# Autodesk Inventor assembly: Final
(part 3 of 3)
- Mate:825: Cap_Platine:3 ↔ din_en_iso_4762_m3x6:5
- Mate:826: Cap_Platine:3 ↔ din_en_iso_4762_m3x6:8
- Mate:827: Cap_Platine:2 ↔ din_en_iso_4762_m3x6:10
- Mate:828: Cap_Platine:2 ↔ din_en_iso_4762_m3x6:15
- Mate:829: Cap_Platine:1 ↔ din_en_iso_4762_m3x6:14
- Mate:830: Cap_Platine:1 ↔ din_en_iso_4762_m3x6:7
- Mate:831: Cap_Platine:6 ↔ din_en_iso_4762_m3x6:3
- Mate:832: Cap_Platine:6 ↔ din_en_iso_4762_m3x6:2
- Mate:833: Cap_Platine:1 ↔ din_en_iso_4762_m3x6:18
- Mate:834: Cap_Platine:4 ↔ din_en_iso_4762_m3x6:16
- Mate:835: Cap_Platine:2 ↔ din_en_iso_4762_m3x6:17
- Mate:836: Cap_Platine:6 ↔ din_en_iso_4762_m3x6:11
- Mate:837: Cap_Platine:3 ↔ din_en_iso_4762_m3x6:13
- Mate:838: Cap_Platine:4 ↔ din_en_iso_4762_m3x6:12
- Mate:839: Cap_Platine:4 ↔ din_en_iso_4762_m3x6:4
- Mate:840: Cap_Platine:3 ↔ din_en_iso_4762_m3x6:8
- Mate:841: Cap_Platine:3 ↔ din_en_iso_4762_m3x6:5
- Mate:842: Secondary:1 ↔ PrimaryCoil:1
- Mate:843: primary_holder:6 ↔ PrimaryCoil:1
- Mate:844: SeitenUnten:2 ↔ Lüfter:4
- Mate:845: SeitenUnten:2 ↔ Lüfter:3
- Mate:846: SeitenUnten:1 ↔ Lüfter:2
- Mate:847: SeitenUnten:1 ↔ Lüfter:1
- Mate:848: SeitenUnten:1 ↔ Lüfter:2
- Mate:849: SeitenUnten:1 ↔ Lüfter:1
- Mate:850: SeitenUnten:2 ↔ Lüfter:3
- Mate:851: SeitenUnten:2 ↔ Lüfter:4
- Mate:852: SeitenUnten:2 ↔ Lüfter:3
- Mate:853: SeitenUnten:2 ↔ Lüfter:4
- Mate:854: SeitenUnten:1 ↔ Lüfter:2
- Mate:855: SeitenUnten:1 ↔ Lüfter:1
- Mate:887: Heatsink:1 ↔ Abstandshalter_5mm:5
- Mate:888: Heatsink:1 ↔ Abstandshalter_5mm:2
- Mate:889: Heatsink:1 ↔ Abstandshalter_5mm:3
- Mate:890: Heatsink:1 ↔ Abstandshalter_5mm:1
- Mate:891: Heatsink:1 ↔ Abstandshalter_5mm:6
- Mate:892: Heatsink:1 ↔ Abstandshalter_5mm:4
- Mate:893: Heatsink:1 ↔ Abstandshalter_5mm:2
- Mate:894: Heatsink:1 ↔ Abstandshalter_5mm:3
- Mate:895: Heatsink:1 ↔ Abstandshalter_5mm:1
- Mate:896: Heatsink:1 ↔ Abstandshalter_5mm:5
- Mate:897: Heatsink:1 ↔ Abstandshalter_5mm:6
- Mate:898: Heatsink:1 ↔ Abstandshalter_5mm:4
- Mate:899: Abstandshalter_5mm:2 ↔ GDT:2
- Mate:900: Abstandshalter_5mm:1 ↔ GDT:1
- Mate:901: Abstandshalter_5mm:4 ↔ GDT:1
- Mate:902: Abstandshalter_5mm:3 ↔ GDT:1
- Mate:903: Abstandshalter_5mm:2 ↔ GDT:2
- Mate:904: Abstandshalter_5mm:6 ↔ GDT:2
- Mate:905: GDT:2 ↔ din_en_iso_4762_m3x6:21
- Mate:906: GDT:2 ↔ din_en_iso_4762_m3x6:20
- Mate:907: GDT:2 ↔ din_en_iso_4762_m3x6:23
- Mate:908: GDT:1 ↔ din_en_iso_4762_m3x6:24
- Mate:909: GDT:1 ↔ din_en_iso_4762_m3x6:19
- Mate:910: GDT:1 ↔ din_en_iso_4762_m3x6:22
- Mate:911: GDT:1 ↔ din_en_iso_4762_m3x6:19
- Mate:912: GDT:1 ↔ din_en_iso_4762_m3x6:22
- Mate:913: GDT:1 ↔ din_en_iso_4762_m3x6:24
- Mate:914: GDT:2 ↔ din_en_iso_4762_m3x6:23
- Mate:915: GDT:2 ↔ din_en_iso_4762_m3x6:21
- Mate:916: GDT:2 ↔ din_en_iso_4762_m3x6:20
- Mate:917: bottom:1 ↔ LogicHolder:1
- Mate:923: SeitenUntenHinten:1 ↔ din_en_iso_4762_m3x10:16
- Mate:924: SeitenUntenHinten:1 ↔ din_en_iso_4762_m3x10:15
- Mate:925: SeitenUntenHinten:1 ↔ din_en_iso_4762_m3x10:16
- Mate:926: SeitenUntenHinten:1 ↔ din_en_iso_4762_m3x10:15
- Mate:927: Netzstecker:1 ↔ din_en_iso_7991_m3x10:4
- Mate:928: Netzstecker:1 ↔ din_en_iso_7991_m3x10:2
- Mate:929: Netzstecker:2 ↔ din_en_iso_7991_m3x10:3
- Mate:930: Netzstecker:2 ↔ din_en_iso_7991_m3x10:1
- Flush:480: Netzstecker:1 ↔ din_en_iso_7991_m3x10:2
- Flush:481: Netzstecker:1 ↔ din_en_iso_7991_m3x10:4
- Flush:482: Netzstecker:2 ↔ din_en_iso_7991_m3x10:1
- Flush:483: Netzstecker:2 ↔ din_en_iso_7991_m3x10:3
- Mate:932: LogicHolder:1 ↔ din_en_iso_7991_m3x10:5
- Mate:933: LogicHolder:1 ↔ din_en_iso_7991_m3x10:6
- Mate:934: bottom:1 ↔ NtHolder:1
- Mate:936: NtHolder:1 ↔ Power_Supply_S_90_18:1
- Mate:937: NtHolder:1 ↔ Power_Supply_S_90_18:1
- Mate:938: NtHolder:1 ↔ din_en_iso_7991_m3x10:8
- Mate:939: NtHolder:1 ↔ din_en_iso_7991_m3x10:7
- Mate:940: NtHolder:1 ↔ din_en_iso_7991_m3x10:9
- Mate:941: NtHolder:1 ↔ din_en_iso_7991_m3x10:10
- Flush:484: LogicHolder:1 ↔ din_en_iso_7991_m3x10:5
- Flush:485: LogicHolder:1 ↔ din_en_iso_7991_m3x10:6
- Flush:486: NtHolder:1 ↔ din_en_iso_7991_m3x10:10
- Flush:487: NtHolder:1 ↔ din_en_iso_7991_m3x10:9
- Flush:488: NtHolder:1 ↔ din_en_iso_7991_m3x10:8
- Flush:489: NtHolder:1 ↔ din_en_iso_7991_m3x10:7
- Mate:942: din_en_iso_7991_m3x10:1 ↔ mutter_din934_m3-6:25
- Mate:943: SeitenUntenHinten:1 ↔ mutter_din934_m3-6:25
- Mate:944: din_en_iso_4762_m3x10:15 ↔ mutter_din934_m3-6:27
- Mate:945: din_en_iso_7991_m3x10:3 ↔ mutter_din934_m3-6:26
- Mate:946: SeitenUntenHinten:1 ↔ mutter_din934_m3-6:26
- Mate:947: Netzfilter:1 ↔ mutter_din934_m3-6:27
- Mate:948: din_en_iso_7991_m3x10:2 ↔ mutter_din934_m3-6:24
- Mate:949: SeitenUntenHinten:1 ↔ mutter_din934_m3-6:24
- Mate:950: din_en_iso_7991_m3x10:4 ↔ mutter_din934_m3-6:28
- Mate:951: din_en_iso_4762_m3x10:16 ↔ mutter_din934_m3-6:23
- Mate:952: Netzfilter:1 ↔ mutter_din934_m3-6:23
- Mate:953: SeitenUntenHinten:1 ↔ mutter_din934_m3-6:28
- Mate:954: Lüfter:2 ↔ din_en_iso_7991_m4x35:16
- Mate:955: Lüfter:1 ↔ din_en_iso_7991_m4x35:9
- Mate:956: Lüfter:1 ↔ din_en_iso_7991_m4x35:10
- Mate:957: Lüfter:2 ↔ din_en_iso_7991_m4x35:11
- Mate:958: Lüfter:2 ↔ din_en_iso_7991_m4x35:12
- Mate:959: Lüfter:2 ↔ din_en_iso_7991_m4x35:13
- Mate:960: Lüfter:1 ↔ din_en_iso_7991_m4x35:14
- Mate:961: Lüfter:1 ↔ din_en_iso_7991_m4x35:15
- Mate:962: Lüfter:4 ↔ din_en_iso_7991_m4x35:1
- Mate:963: Lüfter:4 ↔ din_en_iso_7991_m4x35:2
- Mate:964: Lüfter:4 ↔ din_en_iso_7991_m4x35:3
- Mate:965: Lüfter:4 ↔ din_en_iso_7991_m4x35:4
- Mate:966: Lüfter:3 ↔ din_en_iso_7991_m4x35:5
- Mate:967: Lüfter:3 ↔ din_en_iso_7991_m4x35:6
- Mate:968: Lüfter:3 ↔ din_en_iso_7991_m4x35:7
- Mate:969: Lüfter:3 ↔ din_en_iso_7991_m4x35:8
- Flush:490: SeitenUnten:1 ↔ din_en_iso_7991_m4x35:9
- Flush:491: SeitenUnten:1 ↔ din_en_iso_7991_m4x35:10
- Flush:971: SeitenUnten:1 ↔ din_en_iso_7991_m4x35:11
- Flush:492: SeitenUnten:1 ↔ din_en_iso_7991_m4x35:15
- Flush:493: SeitenUnten:1 ↔ din_en_iso_7991_m4x35:12
- Flush:494: SeitenUnten:1 ↔ din_en_iso_7991_m4x35:13
- Flush:495: SeitenUnten:1 ↔ din_en_iso_7991_m4x35:16
- Flush:496: SeitenUnten:1 ↔ din_en_iso_7991_m4x35:14
- Mate:971: din_en_iso_7991_m4x35:9 ↔ mutter_din934_m4-10:33
- Mate:972: din_en_iso_7991_m4x35:10 ↔ mutter_din934_m4-10:27
- Mate:973: din_en_iso_7991_m4x35:15 ↔ mutter_din934_m4-10:30
- Mate:974: din_en_iso_7991_m4x35:12 ↔ mutter_din934_m4-10:29
- Mate:975: din_en_iso_7991_m4x35:13 ↔ mutter_din934_m4-10:28
- Mate:976: din_en_iso_7991_m4x35:16 ↔ mutter_din934_m4-10:32
- Mate:977: din_en_iso_7991_m4x35:14 ↔ mutter_din934_m4-10:34
- Mate:986: din_en_iso_7991_m4x35:11 ↔ mutter_din934_m4-10:31
- Mate:988: Schalter:1 ↔ Rändelmutter:1
- Mate:989: SeitenUntenVorne:1 ↔ Rändelmutter:1
- Mate:990: Schalter:2 ↔ Rändelmutter:2
- Mate:991: SeitenUntenVorne:1 ↔ Rändelmutter:2
- Flush:972: SeitenUnten:2 ↔ din_en_iso_7991_m4x35:7
- Flush:973: SeitenUnten:2 ↔ din_en_iso_7991_m4x35:8
- Flush:974: SeitenUnten:2 ↔ din_en_iso_7991_m4x35:1
- Flush:975: SeitenUnten:2 ↔ din_en_iso_7991_m4x35:6
- Flush:976: SeitenUnten:2 ↔ din_en_iso_7991_m4x35:2
- Flush:993: SeitenUnten:2 ↔ din_en_iso_7991_m4x35:5
- Mate:992: din_en_iso_7991_m4x35:7 ↔ mutter_din934_m4-10:41
- Mate:994: din_en_iso_7991_m4x35:1 ↔ mutter_din934_m4-10:38
- Mate:996: din_en_iso_7991_m4x35:8 ↔ mutter_din934_m4-10:37
- Mate:997: din_en_iso_7991_m4x35:2 ↔ mutter_din934_m4-10:36
- Mate:1000: din_en_iso_7991_m4x35:6 ↔ mutter_din934_m4-10:42
- Mate:1001: din_en_iso_7991_m4x35:5 ↔ mutter_din934_m4-10:39
- Flush:994: SeitenUnten:2 ↔ din_en_iso_7991_m4x35:4
- Flush:995: SeitenUnten:2 ↔ din_en_iso_7991_m4x35:3
- Mate:1002: din_en_iso_7991_m4x35:3 ↔ mutter_din934_m4-10:40
- Mate:1004: din_en_iso_7991_m4x35:4 ↔ mutter_din934_m4-10:35
- Mate:1007: mid:1 ↔ CT_Holder:2
- Mate:1008: mid:1 ↔ CT_Holder:1
- Angle:7 (0 deg): mid:1 ↔ CT_Holder:1
- Angle:8 (0 deg): mid:1 ↔ CT_Holder:2
- [Mate]: mid:1 ↔ din_en_iso_4762_m3x10:18
- [Mate]: mid:1 ↔ din_en_iso_4762_m3x10:17
- Mate:1011: din_en_iso_4762_m3x10:18 ↔ mutter_din934_m3-6:30
- Mate:1012: mid:1 ↔ mutter_din934_m3-6:30
- Mate:1013: din_en_iso_4762_m3x10:17 ↔ mutter_din934_m3-6:29
- Mate:1014: mid:1 ↔ mutter_din934_m3-6:29
- Mate:1015: Platine_Gleichrichter:1 ↔ din125-1-a_5_3-140_hv:1
- Mate:1016: Cu_Cap:2 ↔ din_en_iso_4762_m5x10:3
- Mate:1017: Cu_Cap:1 ↔ din_en_iso_4762_m5x10:7
- Mate:1018: din125-1-a_5_3-140_hv:6 ↔ din_en_iso_4762_m5x10:2
- Mate:1019: din125-1-a_5_3-140_hv:11 ↔ din_en_iso_4762_m5x10:4
- Mate:1020: din125-1-a_5_3-140_hv:7 ↔ din_en_iso_4762_m5x10:2
- Mate:1021: din125-1-a_5_3-140_hv:5 ↔ din_en_iso_4762_m5x10:4
- Mate:1022: din125-1-a_5_3-140_hv:8 ↔ din_en_iso_4762_m5x10:5
- Mate:1023: din125-1-a_5_3-140_hv:9 ↔ din_en_iso_4762_m5x10:5
- Mate:1024: din125-1-a_5_3-140_hv:10 ↔ din_en_iso_4762_m5x10:8
- Mate:1025: din125-1-a_5_3-140_hv:12 ↔ din_en_iso_4762_m5x10:8
- Mate:1026: din125-1-a_5_3-140_hv:5 ↔ din125-1-a_5_3-140_hv:11
- Mate:1027: Cu_Cap:2 ↔ din125-1-a_5_3-140_hv:11
- Mate:1028: din125-1-a_5_3-140_hv:6 ↔ din125-1-a_5_3-140_hv:7
- Mate:1029: Cu_Cap:1 ↔ din125-1-a_5_3-140_hv:7
- Mate:1030: din125-1-a_5_3-140_hv:8 ↔ din125-1-a_5_3-140_hv:9
- Mate:1031: Cu_Cap:1 ↔ din125-1-a_5_3-140_hv:8
- Mate:1032: din125-1-a_5_3-140_hv:10 ↔ din125-1-a_5_3-140_hv:12
- Mate:1033: Cu_Cap:2 ↔ din125-1-a_5_3-140_hv:12
- Mate:1034: din125-1-a_5_3-140_hv:14 ↔ din_en_iso_4762_m5x10:4
- Mate:1035: din125-1-a_5_3-140_hv:16 ↔ din_en_iso_4762_m5x10:2
- Mate:1036: din125-1-a_5_3-140_hv:5 ↔ din125-1-a_5_3-140_hv:14
- Mate:1037: din125-1-a_5_3-140_hv:6 ↔ din125-1-a_5_3-140_hv:16
- Mate:1038: din125-1-a_5_3-140_hv:13 ↔ din_en_iso_4762_m5x10:5
- Mate:1039: din125-1-a_5_3-140_hv:15 ↔ din_en_iso_4762_m5x10:8
- Mate:1040: din125-1-a_5_3-140_hv:10 ↔ din125-1-a_5_3-140_hv:15
- Mate:1041: din125-1-a_5_3-140_hv:9 ↔ din125-1-a_5_3-140_hv:13
- Mate:1042: Cap:2 ↔ din125-1-a_5_3-140_hv:16
- Mate:1043: din_en_iso_4762_m5x10:7 ↔ mutter_din934_m5-6:11
- Mate:1044: din_en_iso_4762_m5x10:3 ↔ mutter_din934_m5-6:12
- Mate:1045: Cu_Cap:1 ↔ mutter_din934_m5-6:11
- Mate:1046: Cu_Cap:2 ↔ mutter_din934_m5-6:12
- Mate:1047: Lüftergitter:4 ↔ Lüfter:2
- Mate:1048: Lüftergitter:3 ↔ Lüfter:1
- Mate:1049: Lüftergitter:4 ↔ din_en_iso_7991_m4x35:16
- Mate:1050: Lüftergitter:4 ↔ din_en_iso_7991_m4x35:13
- Mate:1051: Lüftergitter:4 ↔ mutter_din934_m4-10:32
- Mate:1052: Lüftergitter:4 ↔ mutter_din934_m4-10:28
- Mate:1053: Lüftergitter:3 ↔ din_en_iso_7991_m4x35:10
- Mate:1054: Lüftergitter:3 ↔ din_en_iso_7991_m4x35:14
- Mate:1055: Lüftergitter:3 ↔ mutter_din934_m4-10:33
- Mate:1056: Lüftergitter:3 ↔ mutter_din934_m4-10:27
- Mate:1057: Lüftergitter:3 ↔ mutter_din934_m4-10:34
- Mate:1058: Lüftergitter:3 ↔ mutter_din934_m4-10:30
- Mate:1059: Lüftergitter:4 ↔ mutter_din934_m4-10:31
- Mate:1060: Lüftergitter:4 ↔ mutter_din934_m4-10:29
- Mate:1061: Lüftergitter:2 ↔ Lüfter:4
- Mate:1062: Lüftergitter:1 ↔ Lüfter:3
- Mate:1063: Lüftergitter:1 ↔ din_en_iso_7991_m4x35:7
- Mate:1064: Lüftergitter:2 ↔ din_en_iso_7991_m4x35:1
- Mate:1065: Lüftergitter:1 ↔ din_en_iso_7991_m4x35:8
- Mate:1066: Lüftergitter:2 ↔ din_en_iso_7991_m4x35:2
- Mate:1067: Lüftergitter:2 ↔ mutter_din934_m4-10:36
- Mate:1068: Lüftergitter:2 ↔ mutter_din934_m4-10:40
- Mate:1069: Lüftergitter:2 ↔ mutter_din934_m4-10:35
- Mate:1070: Lüftergitter:1 ↔ mutter_din934_m4-10:42
- Mate:1071: Lüftergitter:1 ↔ mutter_din934_m4-10:39
- Mate:1072: Lüftergitter:1 ↔ mutter_din934_m4-10:41
- Mate:1073: Lüftergitter:2 ↔ mutter_din934_m4-10:38
- Mate:1074: Lüftergitter:1 ↔ mutter_din934_m4-10:37
- Mate:1075: din_en_iso_4762_m6x10:4 ↔ mutter_din934_m6-6:18
- Mate:1076: din_en_iso_4762_m6x10:2 ↔ mutter_din934_m6-6:17
- Mate:1077: CU5:1 ↔ mutter_din934_m6-6:18
- Mate:1078: cu(:1 ↔ mutter_din934_m6-6:17
- Mate:1079: Gleichrichter:1 ↔ din_en_iso_4762_m4x16:1
- Mate:1080: Gleichrichter:1 ↔ din_en_iso_4762_m4x16:1
- Mate:1081: din125-1-a_3_2-140_hv:13 ↔ din_en_iso_7991_m3x10:7
- Mate:1082: din125-1-a_3_2-140_hv:15 ↔ din_en_iso_7991_m3x10:7
- Mate:1083: din125-1-a_3_2-140_hv:14 ↔ din_en_iso_7991_m3x10:9
- Mate:1084: din125-1-a_3_2-140_hv:16 ↔ din_en_iso_7991_m3x10:9
- Mate:1085: din125-1-a_3_2-140_hv:13 ↔ din125-1-a_3_2-140_hv:15
- Mate:1086: NtHolder:1 ↔ din125-1-a_3_2-140_hv:15
- Mate:1087: din125-1-a_3_2-140_hv:1 ↔ din_en_iso_7991_m3x10:10
- Mate:1088: din125-1-a_3_2-140_hv:10 ↔ din_en_iso_7991_m3x10:10
- Mate:1089: din125-1-a_3_2-140_hv:11 ↔ din_en_iso_7991_m3x10:8
- Mate:1090: din125-1-a_3_2-140_hv:12 ↔ din_en_iso_7991_m3x10:8
- Mate:1091: NtHolder:1 ↔ din125-1-a_3_2-140_hv:11
- Mate:1092: din125-1-a_3_2-140_hv:11 ↔ din125-1-a_3_2-140_hv:12
- Mate:1093: NtHolder:1 ↔ din125-1-a_3_2-140_hv:1
- Mate:1094: din125-1-a_3_2-140_hv:1 ↔ din125-1-a_3_2-140_hv:10
- Mate:1095: NtHolder:1 ↔ din125-1-a_3_2-140_hv:14
- Mate:1096: din125-1-a_3_2-140_hv:14 ↔ din125-1-a_3_2-140_hv:16
- Mate:1097: Power_Supply_S_90_18:1 ↔ din125-1-a_3_2-140_hv:16
- Mate:1098: din125-1-a_3_2-140_hv:8 ↔ din_en_iso_7991_m3x10:6
- Mate:1099: din125-1-a_3_2-140_hv:7 ↔ din_en_iso_7991_m3x10:6
- Mate:1100: din125-1-a_3_2-140_hv:5 ↔ din_en_iso_7991_m3x10:5
- Mate:1101: din125-1-a_3_2-140_hv:6 ↔ din_en_iso_7991_m3x10:5
- Mate:1102: din125-1-a_3_2-140_hv:7 ↔ din125-1-a_3_2-140_hv:8
- Mate:1103: LogicHolder:1 ↔ din125-1-a_3_2-140_hv:8
- Mate:1104: din125-1-a_3_2-140_hv:5 ↔ din125-1-a_3_2-140_hv:6
- Mate:1105: LogicHolder:1 ↔ din125-1-a_3_2-140_hv:6
- Mate:1106: Elektronik_Gehäuse:1 ↔ din125-1-a_3_2-140_hv:5
- Mate:1107: PlexiHalter2:2 ↔ mutter_din934_m3-6:35
- Mate:1108: PlexiHalter2:2 ↔ mutter_din934_m3-6:36
- Mate:1109: PlexiHalter2:2 ↔ mutter_din934_m3-6:37
- Mate:1110: PlexiHalter2:2 ↔ mutter_din934_m3-6:37
- Mate:1111: PlexiHalter2:2 ↔ mutter_din934_m3-6:35
- Mate:1112: PlexiHalter2:2 ↔ mutter_din934_m3-6:36
- Mate:1113: PlexiHalter2:2 ↔ mutter_din934_m3-6:38
- Mate:1114: PlexiHalter2:2 ↔ mutter_din934_m3-6:38
- Mate:1115: PlexiHalter2:2 ↔ din_en_iso_7991_m3x16:8
- Mate:1116: PlexiHalter2:2 ↔ din_en_iso_7991_m3x16:5
- Mate:1117: PlexiHalter2:2 ↔ din_en_iso_7991_m3x16:7
- Mate:1118: PlexiHalter2:2 ↔ din_en_iso_7991_m3x16:6
- Flush:996: Seconday_End_Bottom:1 ↔ din_en_iso_7991_m3x16:6
- Flush:997: Seconday_End_Bottom:1 ↔ din_en_iso_7991_m3x16:5
- Flush:998: Seconday_End_Bottom:1 ↔ din_en_iso_7991_m3x16:7
- Flush:999: Seconday_End_Bottom:1 ↔ din_en_iso_7991_m3x16:8
- Mate:1119: Secondary:1 ↔ PrimaryCoil:2
- Mate:1120: M5 Gewindestange:3 ↔ mutter_din934_m5-6:19
- Mate:1121: bottom:1 ↔ mutter_din934_m5-6:19
- Mate:1122: M5 Gewindestange:2 ↔ mutter_din934_m5-6:18
- Mate:1123: M5 Gewindestange:3 ↔ mutter_din934_m5-6:13
- Mate:1124: M5 Gewindestange:1 ↔ mutter_din934_m5-6:14
- Mate:1125: M5 Gewindestange:1 ↔ mutter_din934_m5-6:20
- Mate:1126: Main:1 ↔ mutter_din934_m5-6:13
- Mate:1127: bottom:1 ↔ mutter_din934_m5-6:18
- Mate:1128: M5 Gewindestange:2 ↔ mutter_din934_m5-6:17
- Mate:1129: M5 Gewindestange:4 ↔ mutter_din934_m5-6:15
- Mate:1130: M5 Gewindestange:4 ↔ mutter_din934_m5-6:16
- Mate:1131: Main:1 ↔ mutter_din934_m5-6:17
- Mate:1132: bottom:1 ↔ mutter_din934_m5-6:15
- Mate:1133: Main:1 ↔ mutter_din934_m5-6:16
- Mate:1134: Main:1 ↔ mutter_din934_m5-6:20
- Mate:1135: bottom:1 ↔ mutter_din934_m5-6:14
- Mate:1136: PrimaryCoil:2
- Mate:1137 (35 mm): Primary:1 ↔ PrimaryCoil:2
